# Autodesk Inventor assembly: Assembly
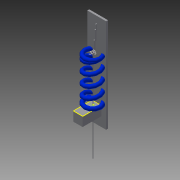
[picture p0: Inventor's stored thumbnail of the model, 180x180]
Saved by Autodesk Inventor 2014 SP1 (Build 180222100, 222)
## iProperties
Created: 2014-01-31
Part Number: Assembly
Document SubType Name: Assembly
Designer: Owner
Author: Owner
## Documents named in this file (8)
- C:\Users\Owner\Documents\GitHub\Team2083-2014-CAD\Winebago Concept\Assembly.iam
- C:\Users\Owner\Documents\GitHub\Team2083-2014-CAD\Winebago Concept\base.ipt
- C:\Users\Owner\Documents\GitHub\Team2083-2014-CAD\Winebago Concept\1.5 in rod.ipt
- C:\Users\Owner\Documents\GitHub\Team2083-2014-CAD\Winebago Concept\3 in bar.ipt
- C:\Users\Owner\Documents\GitHub\Team2083-2014-CAD\Winebago Concept\1 in rod.ipt
- C:\Users\Owner\Documents\GitHub\Team2083-2014-CAD\Winebago Concept\5 in bar.ipt
- C:\Users\Owner\Documents\GitHub\Team2083-2014-CAD\Winebago Concept\right angle rod holder.ipt
- C:\Users\Owner\Documents\GitHub\Team2083-2014-CAD\Winebago Concept\50 in rod.ipt
## Components (10 placed, 7 different names)
1. base:1 — Insert:1, Mate:1
2. 1.5 in rod:1 — Insert:1, Insert:2, Rotation:1
3. 3 in bar:1 — Insert:2, Insert:3, Insert:4, Rotation:1
4. 1 in rod:1 — Insert:3, Insert:5
5. 1 in rod:2 — Insert:4
6. 1 in rod:3 — Insert:6, Insert:7
7. 5 in bar:1 — Insert:5, Insert:6
8. 5 in bar:2 — Insert:7, Insert:8
9. right angle rod holder:1 — Insert:8, Mate:2, Insert:9
10. 50 in rod:1 — Mate:1, Mate:2, Insert:9
## Relationships (12: Insert 9, Mate 2, RelateRotation 1)
- Insert:1: base:1 ↔ 1.5 in rod:1
- Insert:2: 1.5 in rod:1 ↔ 3 in bar:1
- Insert:3: 3 in bar:1 ↔ 1 in rod:1
- Insert:4: 3 in bar:1 ↔ 1 in rod:2
- Insert:5: 1 in rod:1 ↔ 5 in bar:1
- Insert:6: 1 in rod:3 ↔ 5 in bar:1
- Insert:7: 1 in rod:3 ↔ 5 in bar:2
- Insert:8: 5 in bar:2 ↔ right angle rod holder:1
- Mate:1: base:1 ↔ 50 in rod:1
- Mate:2: right angle rod holder:1 ↔ 50 in rod:1
- Rotation:1 [RelateRotation] (1 ul): 1.5 in rod:1 ↔ 3 in bar:1
- Insert:9: right angle rod holder:1 ↔ 50 in rod:1
